# Autodesk Inventor assembly: Wheel Orientation
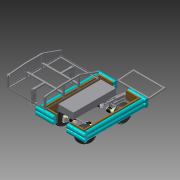
[picture p0: Inventor's stored thumbnail of the model, 180x180]
Saved by Autodesk Inventor 2015 (Build 190159000, 159)
## iProperties
Created: 2016-01-19
Part Number: Wheel Orientation
Document SubType Name: Assembly
Designer: sethbattis
Author: sethbattis
## Documents named in this file (9)
- \\area51\team3566\cad\FRC 2016\Space Claims.iam
- \\area51\team3566\cad\FRC 2016\Wheelbase.ipt
- \\area51\team3566\cad\FRC 2016\Basic Frame.ipt
- \\area51\team3566\cad\FRC 2016\Snow Blower Tire with Gear Box and Mini-CIM.iam
- \\area51\team3566\cad\FRC 2016\Snow Blower Tire with Gear Box and Mini-CIM_MIR.iam
- \\area51\team3566\cad\FRC 2016\Side Bumper.ipt
- \\area51\team3566\cad\FRC 2016\Prow rev2.ipt
- \\area51\team3566\cad\FRC 2016\Catapult Base.ipt
- \\area51\team3566\cad\FRC 2016\Chassis.ipt
## Components (11 placed, 8 different names)
1. Basic Frame:1 — Flush:1, Rigid:1, Mate:13, Flush:16, Flush:17, Mate:14, Flush:18, Flush:19, Mate:19, Mate:20
2. Wheelbase:1 — Flush:1, Rigid:1, Rotational:1, Rotational:2, Rotational:3, Rotational:4, Mate:21, Mate:23, Mate:24
3. Prow rev2:1 — Mate:22, Mate:23, Mate:24
4. Catapult Base:1
5. Chassis:1
6. Side Bumper:2 — Mate:14, Flush:18, Flush:19
7. Side Bumper:1 — Mate:13, Flush:16, Flush:17
8. Snow Blower Tire with Gear Box and Mini-CIM:1 [sub-assembly] — Rotational:1
9. Snow Blower Tire with Gear Box and Mini-CIM:2 [sub-assembly] — Rotational:2
10. Snow Blower Tire with Gear Box and Mini-CIM_MIR:1 [sub-assembly] — Rotational:4
11. Snow Blower Tire with Gear Box and Mini-CIM_MIR:2 [sub-assembly] — Rotational:3
## Relationships (18: Mate 8, Flush 5, RevoluteJoint 4, WeldJoint 1)
- Flush:1: Basic Frame:1 ↔ Wheelbase:1
- Rigid:1 [WeldJoint]: Basic Frame:1 ↔ Wheelbase:1
- Rotational:1 [RevoluteJoint]: Wheelbase:1 ↔ Snow Blower Tire with Gear Box and Mini-CIM:1
- Rotational:2 [RevoluteJoint]: Wheelbase:1 ↔ Snow Blower Tire with Gear Box and Mini-CIM:2
- Rotational:3 [RevoluteJoint]: Wheelbase:1 ↔ Snow Blower Tire with Gear Box and Mini-CIM_MIR:2
- Rotational:4 [RevoluteJoint]: Wheelbase:1 ↔ Snow Blower Tire with Gear Box and Mini-CIM_MIR:1
- Mate:13: Basic Frame:1 ↔ Side Bumper:1
- Flush:16: Basic Frame:1 ↔ Side Bumper:1
- Flush:17: Basic Frame:1 ↔ Side Bumper:1
- Mate:14: Basic Frame:1 ↔ Side Bumper:2
- Flush:18: Basic Frame:1 ↔ Side Bumper:2
- Flush:19: Basic Frame:1 ↔ Side Bumper:2
- Mate:19: Basic Frame:1
- Mate:20: Basic Frame:1
- Mate:21: Wheelbase:1
- Mate:22: Prow rev2:1
- Mate:23: Wheelbase:1 ↔ Prow rev2:1
- Mate:24: Wheelbase:1 ↔ Prow rev2:1
